# Autodesk Inventor assembly: FinalGantry
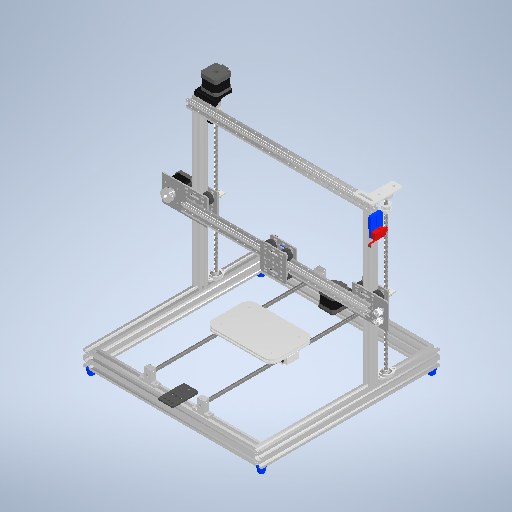
[picture p0: Inventor's stored thumbnail of the model, 512x512]
Saved by Autodesk Inventor 2025.2 (Build 292293000, 293)
## iProperties
Created: 2025-07-17
Part Number: FinalGantry
Document SubType Name: Assembly
Designer: Simon
Author: Simon
## Documents named in this file (34)
- C:\Users\Simon\Projects\Hydrogel-3D-Printer\Hardware\Bioprinter Machine Design\Final System\Final Gantry\FinalGantry.iam
- C:\Users\Simon\Projects\Hydrogel-3D-Printer\Hardware\Bioprinter Machine Design\Final System\Final Gantry\2040_AluminimProfile_410.ipt
- C:\Users\Simon\Projects\Hydrogel-3D-Printer\Hardware\Bioprinter Machine Design\Final System\Final Gantry\2040_AluminimProfile_450.ipt
- C:\Users\Simon\Projects\Hydrogel-3D-Printer\Hardware\Bioprinter Machine Design\Final System\Final Gantry\2020_AluminiumProfile_380.ipt
- C:\Users\Simon\Projects\Hydrogel-3D-Printer\Hardware\Bioprinter Machine Design\Final System\Final Gantry\2020_AluminiumProfile_465.ipt
- C:\Users\Simon\Projects\Hydrogel-3D-Printer\Hardware\Bioprinter Machine Design\PartsFolder\bracket nema 17.ipt
- C:\Users\Simon\Projects\Hydrogel-3D-Printer\Hardware\Bioprinter Machine Design\PartsFolder\Pillow Block Bearing 1\Zinc Alloy Pillow Block Flange Bearing KFL08 ID-8mm.iam
- C:\Users\Simon\Projects\Hydrogel-3D-Printer\Hardware\Bioprinter Machine Design\PartsFolder\Stepper_17HS4401.ipt
- C:\Users\Simon\Projects\Hydrogel-3D-Printer\Hardware\Bioprinter Machine Design\PartsFolder\Flexible Coupling 5,8.ipt
- C:\Users\Simon\Projects\Hydrogel-3D-Printer\Hardware\Bioprinter Machine Design\Final System\Final Gantry\TR8x8-4_LeadScrew_385.ipt
- C:\Users\Simon\Projects\Hydrogel-3D-Printer\Hardware\Bioprinter Machine Design\PartsFolder\TR8x8-4_Nut.ipt
- C:\Users\Simon\Projects\Hydrogel-3D-Printer\Hardware\Bioprinter Machine Design\PartsFolder\Nema 17 Flat Mount.ipt
- C:\Users\Simon\Projects\Hydrogel-3D-Printer\Hardware\Bioprinter Machine Design\PartsFolder\GT2_20T_5.ipt
- C:\Users\Simon\Projects\Hydrogel-3D-Printer\Hardware\Bioprinter Machine Design\PartsFolder\SK8_LinearShaftSupport.ipt
- C:\Users\Simon\Projects\Hydrogel-3D-Printer\Hardware\Bioprinter Machine Design\Final System\Final Gantry\SteelShaft_444mm.ipt
- C:\Users\Simon\Projects\Hydrogel-3D-Printer\Hardware\Bioprinter Machine Design\PartsFolder\SC8UU\SC8UU.iam
- C:\Users\Simon\Projects\Hydrogel-3D-Printer\Hardware\Bioprinter Machine Design\PartsFolder\POM Wheel v2.ipt
- C:\Users\Simon\Projects\Hydrogel-3D-Printer\Hardware\Bioprinter Machine Design\PartsFolder\Carriage Plate v1.ipt
- C:\Users\Simon\Projects\Hydrogel-3D-Printer\Hardware\Bioprinter Machine Design\PartsFolder\Spacer v2.ipt
- C:\Users\Simon\Projects\Hydrogel-3D-Printer\Hardware\Bioprinter Machine Design\Final System\Final Gantry\2020_AluminiumProfile_460.ipt
- C:\Users\Simon\Projects\Hydrogel-3D-Printer\Hardware\Bioprinter Machine Design\Final System\Final Gantry\LeadCarriageConnector.ipt
- C:\Users\Simon\Projects\Hydrogel-3D-Printer\Hardware\Bioprinter Machine Design\Final System\Final Gantry\CarriagePlate_Motor.ipt
- C:\Users\Simon\Projects\Hydrogel-3D-Printer\Hardware\Bioprinter Machine Design\Final System\Final Gantry\CarriagePlate_Idler.ipt
- C:\Users\Simon\Projects\Hydrogel-3D-Printer\Hardware\Bioprinter Machine Design\PartsFolder\GT2_20T_Toothed_Idler_5.ipt
- C:\Users\Simon\Projects\Hydrogel-3D-Printer\Hardware\Bioprinter Machine Design\PartsFolder\Idler Pulley Plate.ipt
- C:\Users\Simon\Projects\Hydrogel-3D-Printer\Hardware\Bioprinter Machine Design\Final System\Final Gantry\BedHeatSink.ipt
- C:\Users\Simon\Projects\Hydrogel-3D-Printer\Hardware\Bioprinter Machine Design\PartsFolder\PeltierTEC1_12706.ipt
- C:\Users\Simon\Projects\Hydrogel-3D-Printer\Hardware\Bioprinter Machine Design\Final System\Final Gantry\ColdPlate.ipt
- C:\Users\Simon\Projects\Hydrogel-3D-Printer\Hardware\Bioprinter Machine Design\Final System\Final Gantry\LeadScrewEndMount.ipt
- C:\Users\Simon\Projects\Hydrogel-3D-Printer\Hardware\Bioprinter Machine Design\PartsFolder\GT2_36T_5.ipt
- C:\Users\Simon\Projects\Hydrogel-3D-Printer\Hardware\Bioprinter Machine Design\PartsFolder\GT2_30T_8.ipt
- C:\Users\Simon\Projects\Hydrogel-3D-Printer\Hardware\Bioprinter Machine Design\Gantry Concept 3\LimitSwitch.ipt
- C:\Users\Simon\Projects\Hydrogel-3D-Printer\Hardware\Bioprinter Machine Design\PartsFolder\Limit Switch\LimitSwitchPart.iam
- C:\Users\Simon\Projects\Hydrogel-3D-Printer\Hardware\Bioprinter Machine Design\Final System\Final Gantry\PrinterFeet.ipt
## Components (96 placed, 33 different names)
1. 2040_AluminimProfile_410:1 — Mate:6, Mate:7, Flush:1, Mate:10, Mate:38, Mate:39, Flush:16, Flush:17, Flush:56, Mate:146, Flush:61, Mate:150, Mate:179, Mate:185
2. 2040_AluminimProfile_450:1 — Mate:1, Mate:2, Mate:4, Mate:7, Flush:1, Mate:9, Flush:2, Mate:11, Flush:3, Mate:14, Mate:16, Angle:2, Mate:183, Mate:186
3. 2040_AluminimProfile_410:2 — Mate:8, Mate:9, Flush:2, Mate:31, Mate:32, Mate:36, Mate:37, Flush:14, Flush:15, Mate:182, Mate:184
4. 2040_AluminimProfile_450:2 — Mate:3, Mate:5, Mate:10, Mate:12, Flush:4, Mate:15, Mate:17, Angle:3, Flush:51, Flush:57, Mate:180, Mate:181, Mate:187
5. 2020_AluminiumProfile_380:1 — Mate:11, Flush:3, Flush:7, Mate:82, Flush:41
6. 2020_AluminiumProfile_380:2 — Mate:12, Flush:4, Mate:13, Flush:5, Flush:6, Mate:83, Mate:98, Flush:56, Mate:171, Flush:68
7. 2020_AluminiumProfile_465:1 — Mate:13, Flush:5, Flush:6, Flush:7, Mate:18, Flush:9, Flush:59, Mate:160, Flush:64, Flush:65
8. bracket nema 17:1 — Mate:18, Mate:19, Flush:9, Mate:20, Mate:21, Angle:1
9. Zinc Alloy Pillow Block Flange Bearing KFL08 ID-8mm:1 [sub-assembly] — Mate:14, Mate:16, Flush:8, Mate:19, Mate:23
10. Zinc Alloy Pillow Block Flange Bearing KFL08 ID-8mm:2 [sub-assembly] — Mate:15, Mate:17, Flush:8, Mate:24, Mate:145
11. Stepper_17HS4401:1 — Mate:20, Mate:21, Angle:1, Mate:22, Flush:10, Mate:25
12. Flexible Coupling 5,8:1 — Mate:22, Flush:10, Mate:170
13. TR8x8-4_LeadScrew_385:1 — Mate:23, Flush:11, Mate:25, Mate:26, Mate:169
14. TR8x8-4_LeadScrew_385:2 — Mate:24, Flush:11, Mate:27, Mate:144, Mate:168
15. TR8x8-4_Nut:1 — Mate:26, Flush:12, Angle:5, Mate:90
16. TR8x8-4_Nut:2 — Mate:27, Flush:12, Angle:4
17. Nema 17 Flat Mount:1 — Mate:31, Mate:32, Mate:33, Mate:34, Flush:60, Angle:11
18. Stepper_17HS4401:2 — Mate:33, Mate:34, Mate:35, Angle:11
19. GT2_20T_5:1 — Mate:35, Flush:62
20. SK8_LinearShaftSupport:1 — Mate:36, Flush:14, Mate:40
21. SK8_LinearShaftSupport:2 — Mate:37, Flush:15, Mate:41
22. SK8_LinearShaftSupport:3 — Mate:38, Flush:17, Mate:40, Mate:42, Flush:18
23. SK8_LinearShaftSupport:4 — Mate:39, Flush:16, Mate:41, Mate:43, Flush:19
24. SteelShaft_444mm:1 — Mate:42, Flush:18, Mate:44
25. SteelShaft_444mm:2 — Mate:43, Flush:19, Mate:45
26. SC8UU:1 [sub-assembly] — Mate:44, Angle:2, Flush:20, Flush:58, Mate:147
27. SC8UU:2 [sub-assembly] — Mate:45, Angle:3, Flush:20, Mate:143, Mate:148, Mate:149
28. POM Wheel v2:1 — Mate:54, Flush:27, Mate:62, Mate:99
29. POM Wheel v2:2 — Flush:27, Flush:28, Mate:61, Mate:82, Mate:105
30. POM Wheel v2:3 — Flush:28, Flush:29, Mate:104
31. POM Wheel v2:4 — Flush:29, Mate:103
32. Carriage Plate v1:2 — Mate:54, Mate:56, Mate:57, Mate:58, Mate:59, Mate:60, Mate:85, Mate:87, Mate:89, Flush:40, Flush:41
33. Spacer v2:1 — Flush:24, Mate:62, Mate:99
34. Spacer v2:2 — Flush:24, Flush:25, Mate:100, Mate:105, Mate:130
35. Spacer v2:3 — Flush:25, Flush:26, Mate:102
36. Spacer v2:4 — Flush:26, Mate:101, Mate:129, Mate:131
37. Spacer v2:5 — Mate:56, Flush:21
38. Spacer v2:6 — Mate:57, Flush:21, Flush:22, Mate:60, Mate:61, Mate:100
39. Spacer v2:7 — Mate:58, Flush:22, Flush:23, Mate:102, Mate:104
40. Spacer v2:8 — Mate:59, Flush:23, Mate:101, Mate:103
41. POM Wheel v2:5 — Mate:91
42. POM Wheel v2:6 — Mate:83, Mate:97
43. POM Wheel v2:7 — Mate:95
44. POM Wheel v2:8 — Mate:96
45. Carriage Plate v1:4 — Mate:84, Mate:86, Mate:88, Mate:98, Flush:40
46. Spacer v2:9 — Mate:91, Mate:137
47. Spacer v2:10 — Mate:93, Mate:138
48. Spacer v2:11 — Mate:94, Mate:95, Mate:136
49. Spacer v2:12 — Mate:92
50. Spacer v2:13
51. Spacer v2:14 — Mate:93, Mate:97
52. Spacer v2:15 — Mate:94
53. Spacer v2:16 — Mate:92, Mate:96
54. 2020_AluminiumProfile_460:1 — Flush:51, Flush:52, Flush:53, Mate:132, Flush:54
55. LeadCarriageConnector:1 — Mate:84, Mate:86, Mate:88, Angle:4
56. LeadCarriageConnector:2 — Mate:85, Mate:87, Mate:89, Angle:5, Mate:90
57. POM Wheel v2:9 — Flush:52
58. POM Wheel v2:10
59. POM Wheel v2:11
60. POM Wheel v2:12
61. Carriage Plate v1:5 — Flush:53, Mate:172, Angle:8, Mate:173
62. Spacer v2:17 — Mate:127
63. Spacer v2:18 — Mate:128
64. Spacer v2:19 — Mate:126
65. Spacer v2:20
66. Spacer v2:21
67. Spacer v2:22
68. Spacer v2:23
69. Spacer v2:24
70. Carriage Plate v1:6 — Mate:126, Mate:127, Mate:128
71. Stepper_17HS4401:3 — Mate:133, Mate:134, Angle:6, Mate:167
72. CarriagePlate_Motor:1 — Mate:129, Mate:130, Mate:131, Mate:132, Flush:54, Mate:133, Mate:134, Angle:6
73. CarriagePlate_Idler:1 — Mate:136, Mate:137, Mate:138, Mate:141, Mate:161, Mate:165, Mate:166
74. GT2_20T_Toothed_Idler_5:1 — Mate:142, Mate:162, Flush:66
75. Spacer v2:25 — Mate:141, Mate:142, Mate:161, Mate:162
76. Zinc Alloy Pillow Block Flange Bearing KFL08 ID-8mm:3 [sub-assembly] — Mate:144, Flush:59, Mate:145
77. Idler Pulley Plate:1 — Mate:146, Flush:60, Flush:61, Mate:150, Mate:151, Mate:157, Mate:158
78. BedHeatSink:1 — Mate:147, Mate:148, Mate:149, Mate:152, Angle:7, Mate:153, Flush:63, Mate:154, Mate:155
79. GT2_20T_Toothed_Idler_5:2 — Mate:151, Flush:62, Mate:159
80. PeltierTEC1_12706:1 — Mate:152, Angle:7, Mate:153, Flush:63, Mate:156
81. ColdPlate:1 — Mate:154, Mate:155, Mate:156
82. Spacer v2:26 — Mate:157, Mate:158, Mate:159
83. LeadScrewEndMount:1 — Mate:160, Flush:64, Flush:65, Mate:176
84. GT2_20T_Toothed_Idler_5:3 — Mate:166
85. Spacer v2:27 — Mate:165
86. GT2_36T_5:1 — Mate:167, Flush:66
87. GT2_30T_8:1 — Mate:169, Flush:67, Mate:170
88. GT2_30T_8:2 — Mate:168, Flush:67
89. LimitSwitch:1 — Mate:171, Flush:68, Mate:176, Mate:177, Angle:10, Mate:178
90. LimitSwitch:2 — Mate:172, Angle:8, Mate:173, Mate:174, Angle:9, Mate:175
91. LimitSwitchPart:1 [sub-assembly] — Mate:177, Angle:10, Mate:178
92. LimitSwitchPart:2 [sub-assembly] — Mate:174, Angle:9, Mate:175
93. PrinterFeet:1 — Flush:70, Mate:183, Mate:184
94. PrinterFeet:2 — Flush:69, Flush:70, Mate:185, Mate:186
95. PrinterFeet:3 — Flush:69, Flush:71, Mate:181, Mate:182
96. PrinterFeet:4 — Flush:71, Mate:179, Mate:180, Mate:187
## Relationships (235: Mate 156, Flush 68, Angle 11)
- Mate:1: 2040_AluminimProfile_450:1
- Mate:2: 2040_AluminimProfile_450:1
- Mate:3: 2040_AluminimProfile_450:2
- Mate:4: 2040_AluminimProfile_450:1
- Mate:5: 2040_AluminimProfile_450:2
- Mate:6: 2040_AluminimProfile_410:1
- Mate:7: 2040_AluminimProfile_410:1 ↔ 2040_AluminimProfile_450:1
- Flush:1: 2040_AluminimProfile_410:1 ↔ 2040_AluminimProfile_450:1
- Mate:8: 2040_AluminimProfile_410:2
- Mate:9: 2040_AluminimProfile_450:1 ↔ 2040_AluminimProfile_410:2
- Flush:2: 2040_AluminimProfile_450:1 ↔ 2040_AluminimProfile_410:2
- Mate:10: 2040_AluminimProfile_410:1 ↔ 2040_AluminimProfile_450:2
- Mate:11: 2040_AluminimProfile_450:1 ↔ 2020_AluminiumProfile_380:1
- Mate:12: 2040_AluminimProfile_450:2 ↔ 2020_AluminiumProfile_380:2
- Flush:3: 2040_AluminimProfile_450:1 ↔ 2020_AluminiumProfile_380:1
- Flush:4: 2040_AluminimProfile_450:2 ↔ 2020_AluminiumProfile_380:2
- Mate:13: 2020_AluminiumProfile_380:2 ↔ 2020_AluminiumProfile_465:1
- Flush:5: 2020_AluminiumProfile_380:2 ↔ 2020_AluminiumProfile_465:1
- Flush:6: 2020_AluminiumProfile_380:2 ↔ 2020_AluminiumProfile_465:1
- Flush:7: 2020_AluminiumProfile_380:1 ↔ 2020_AluminiumProfile_465:1
- Mate:14: 2040_AluminimProfile_450:1 ↔ Zinc Alloy Pillow Block Flange Bearing KFL08 ID-8mm:1
- Mate:15: 2040_AluminimProfile_450:2 ↔ Zinc Alloy Pillow Block Flange Bearing KFL08 ID-8mm:2
- Mate:16: 2040_AluminimProfile_450:1 ↔ Zinc Alloy Pillow Block Flange Bearing KFL08 ID-8mm:1
- Mate:17: 2040_AluminimProfile_450:2 ↔ Zinc Alloy Pillow Block Flange Bearing KFL08 ID-8mm:2
- Flush:8: Zinc Alloy Pillow Block Flange Bearing KFL08 ID-8mm:1 ↔ Zinc Alloy Pillow Block Flange Bearing KFL08 ID-8mm:2
- Mate:18: 2020_AluminiumProfile_465:1 ↔ bracket nema 17:1
- Mate:19: bracket nema 17:1 ↔ Zinc Alloy Pillow Block Flange Bearing KFL08 ID-8mm:1
- Flush:9 (-10 mm): 2020_AluminiumProfile_465:1 ↔ bracket nema 17:1
- Mate:20: bracket nema 17:1 ↔ Stepper_17HS4401:1
- Mate:21: bracket nema 17:1 ↔ Stepper_17HS4401:1
- Angle:1 (0 deg): bracket nema 17:1 ↔ Stepper_17HS4401:1
- Mate:22: Stepper_17HS4401:1 ↔ Flexible Coupling 5,8:1
- Flush:10 (5 mm): Stepper_17HS4401:1 ↔ Flexible Coupling 5,8:1
- Mate:23: Zinc Alloy Pillow Block Flange Bearing KFL08 ID-8mm:1 ↔ TR8x8-4_LeadScrew_385:1
- Mate:24: Zinc Alloy Pillow Block Flange Bearing KFL08 ID-8mm:2 ↔ TR8x8-4_LeadScrew_385:2
- Flush:11: TR8x8-4_LeadScrew_385:1 ↔ TR8x8-4_LeadScrew_385:2
- Mate:25: Stepper_17HS4401:1 ↔ TR8x8-4_LeadScrew_385:1
- Mate:26: TR8x8-4_LeadScrew_385:1 ↔ TR8x8-4_Nut:1
- Mate:27: TR8x8-4_LeadScrew_385:2 ↔ TR8x8-4_Nut:2
- Flush:12: TR8x8-4_Nut:1 ↔ TR8x8-4_Nut:2
- Mate:31: 2040_AluminimProfile_410:2 ↔ Nema 17 Flat Mount:1
- Mate:32: 2040_AluminimProfile_410:2 ↔ Nema 17 Flat Mount:1
- Mate:33: Nema 17 Flat Mount:1 ↔ Stepper_17HS4401:2
- Mate:34: Nema 17 Flat Mount:1 ↔ Stepper_17HS4401:2
- Mate:35: Stepper_17HS4401:2 ↔ GT2_20T_5:1
- Mate:36: 2040_AluminimProfile_410:2 ↔ SK8_LinearShaftSupport:1
- Mate:37: 2040_AluminimProfile_410:2 ↔ SK8_LinearShaftSupport:2
- Mate:38: 2040_AluminimProfile_410:1 ↔ SK8_LinearShaftSupport:3
- Mate:39: 2040_AluminimProfile_410:1 ↔ SK8_LinearShaftSupport:4
- Flush:14: 2040_AluminimProfile_410:2 ↔ SK8_LinearShaftSupport:1
- Flush:15: 2040_AluminimProfile_410:2 ↔ SK8_LinearShaftSupport:2
- Flush:16: 2040_AluminimProfile_410:1 ↔ SK8_LinearShaftSupport:4
- Flush:17: 2040_AluminimProfile_410:1 ↔ SK8_LinearShaftSupport:3
- Mate:40: SK8_LinearShaftSupport:1 ↔ SK8_LinearShaftSupport:3
- Mate:41: SK8_LinearShaftSupport:2 ↔ SK8_LinearShaftSupport:4
- Mate:42: SK8_LinearShaftSupport:3 ↔ SteelShaft_444mm:1
- Mate:43: SK8_LinearShaftSupport:4 ↔ SteelShaft_444mm:2
- Flush:18: SK8_LinearShaftSupport:3 ↔ SteelShaft_444mm:1
- Flush:19: SK8_LinearShaftSupport:4 ↔ SteelShaft_444mm:2
- Mate:44: SteelShaft_444mm:1 ↔ SC8UU:1
- Mate:45: SteelShaft_444mm:2 ↔ SC8UU:2
- Angle:2 (0 deg): 2040_AluminimProfile_450:1 ↔ SC8UU:1
- Angle:3 (0 deg): 2040_AluminimProfile_450:2 ↔ SC8UU:2
- Flush:20: SC8UU:1 ↔ SC8UU:2
- Mate:54: POM Wheel v2:1 ↔ Carriage Plate v1:2
- Mate:56: Carriage Plate v1:2 ↔ Spacer v2:5
- Mate:57: Carriage Plate v1:2 ↔ Spacer v2:6
- Mate:58: Carriage Plate v1:2 ↔ Spacer v2:7
- Mate:59: Carriage Plate v1:2 ↔ Spacer v2:8
- Flush:21: Spacer v2:5 ↔ Spacer v2:6
- Flush:22: Spacer v2:6 ↔ Spacer v2:7
- Flush:23: Spacer v2:7 ↔ Spacer v2:8
- Mate:60: Carriage Plate v1:2 ↔ Spacer v2:6
- Flush:24: Spacer v2:1 ↔ Spacer v2:2
- Flush:25: Spacer v2:2 ↔ Spacer v2:3
- Flush:26: Spacer v2:3 ↔ Spacer v2:4
- Flush:27: POM Wheel v2:1 ↔ POM Wheel v2:2
- Flush:28: POM Wheel v2:2 ↔ POM Wheel v2:3
- Flush:29: POM Wheel v2:3 ↔ POM Wheel v2:4
- Mate:61: POM Wheel v2:2 ↔ Spacer v2:6
- Mate:62: POM Wheel v2:1 ↔ Spacer v2:1
- [Mate]: POM Wheel v2:5 ↔ Carriage Plate v1:4
- [Mate]: Carriage Plate v1:4 ↔ Spacer v2:13
- [Mate]: Carriage Plate v1:4 ↔ Spacer v2:14
- [Mate]: Carriage Plate v1:4 ↔ Spacer v2:15
- [Mate]: Carriage Plate v1:4 ↔ Spacer v2:16
- [Flush]: Spacer v2:13 ↔ Spacer v2:14
- [Flush]: Spacer v2:14 ↔ Spacer v2:15
- [Flush]: Spacer v2:15 ↔ Spacer v2:16
- [Mate]: Carriage Plate v1:4 ↔ Spacer v2:14
- [Flush]: Spacer v2:9 ↔ Spacer v2:10
- [Flush]: Spacer v2:10 ↔ Spacer v2:11
- [Flush]: Spacer v2:11 ↔ Spacer v2:12
- [Flush]: POM Wheel v2:5 ↔ POM Wheel v2:6
- [Flush]: POM Wheel v2:6 ↔ POM Wheel v2:7
- [Flush]: POM Wheel v2:7 ↔ POM Wheel v2:8
- [Mate]: POM Wheel v2:6 ↔ Spacer v2:14
- [Mate]: POM Wheel v2:5 ↔ Spacer v2:9
- Mate:82: 2020_AluminiumProfile_380:1 ↔ POM Wheel v2:2
- Mate:83: 2020_AluminiumProfile_380:2 ↔ POM Wheel v2:6
- Mate:84: Carriage Plate v1:4 ↔ LeadCarriageConnector:1
- Mate:85: Carriage Plate v1:2 ↔ LeadCarriageConnector:2
- Mate:86: Carriage Plate v1:4 ↔ LeadCarriageConnector:1
- Mate:87: Carriage Plate v1:2 ↔ LeadCarriageConnector:2
- Mate:88: Carriage Plate v1:4 ↔ LeadCarriageConnector:1
- Mate:89: Carriage Plate v1:2 ↔ LeadCarriageConnector:2
- Angle:4 (0 deg): TR8x8-4_Nut:2 ↔ LeadCarriageConnector:1
- Angle:5 (0 deg): TR8x8-4_Nut:1 ↔ LeadCarriageConnector:2
- Mate:90: TR8x8-4_Nut:1 ↔ LeadCarriageConnector:2
- Mate:91: POM Wheel v2:5 ↔ Spacer v2:9
- Mate:92: Spacer v2:12 ↔ Spacer v2:16
- Mate:93: Spacer v2:10 ↔ Spacer v2:14
- Mate:94: Spacer v2:11 ↔ Spacer v2:15
- Mate:95: POM Wheel v2:7 ↔ Spacer v2:11
- Mate:96: POM Wheel v2:8 ↔ Spacer v2:16
- Mate:97: POM Wheel v2:6 ↔ Spacer v2:14
- Mate:98: 2020_AluminiumProfile_380:2 ↔ Carriage Plate v1:4
- Flush:40: Carriage Plate v1:2 ↔ Carriage Plate v1:4
- Mate:99: POM Wheel v2:1 ↔ Spacer v2:1
- Mate:100: Spacer v2:2 ↔ Spacer v2:6
- Mate:101: Spacer v2:4 ↔ Spacer v2:8
- Mate:102: Spacer v2:3 ↔ Spacer v2:7
- Mate:103: POM Wheel v2:4 ↔ Spacer v2:8
- Mate:104: POM Wheel v2:3 ↔ Spacer v2:7
- Mate:105: POM Wheel v2:2 ↔ Spacer v2:2
- Flush:41: 2020_AluminiumProfile_380:1 ↔ Carriage Plate v1:2
- [Mate]: POM Wheel v2:9 ↔ Carriage Plate v1:5
- [Mate]: Carriage Plate v1:5 ↔ Spacer v2:21
- [Mate]: Carriage Plate v1:5 ↔ Spacer v2:22
- [Mate]: Carriage Plate v1:5 ↔ Spacer v2:23
- [Mate]: Carriage Plate v1:5 ↔ Spacer v2:24
- [Flush]: Spacer v2:21 ↔ Spacer v2:22
- [Flush]: Spacer v2:22 ↔ Spacer v2:23
- [Flush]: Spacer v2:23 ↔ Spacer v2:24
- [Mate]: Carriage Plate v1:5 ↔ Spacer v2:22
- [Flush]: Spacer v2:17 ↔ Spacer v2:18
- [Flush]: Spacer v2:18 ↔ Spacer v2:19
- [Flush]: Spacer v2:19 ↔ Spacer v2:20
- [Flush]: POM Wheel v2:9 ↔ POM Wheel v2:10
- [Flush]: POM Wheel v2:10 ↔ POM Wheel v2:11
- [Flush]: POM Wheel v2:11 ↔ POM Wheel v2:12
- [Mate]: POM Wheel v2:10 ↔ Spacer v2:22
- [Mate]: POM Wheel v2:9 ↔ Spacer v2:17
- [Mate]: POM Wheel v2:9 ↔ Spacer v2:17
- [Mate]: Spacer v2:18 ↔ Spacer v2:22
- [Mate]: Spacer v2:20 ↔ Spacer v2:24
- [Mate]: Spacer v2:19 ↔ Spacer v2:23
- [Mate]: POM Wheel v2:12 ↔ Spacer v2:24
- [Mate]: POM Wheel v2:11 ↔ Spacer v2:23
- [Mate]: POM Wheel v2:10 ↔ Spacer v2:18
- Flush:51 (225 mm): 2040_AluminimProfile_450:2 ↔ 2020_AluminiumProfile_460:1
- Flush:52: 2020_AluminiumProfile_460:1 ↔ POM Wheel v2:9
- Flush:53: 2020_AluminiumProfile_460:1 ↔ Carriage Plate v1:5
- Mate:126: Spacer v2:19 ↔ Carriage Plate v1:6
- Mate:127: Spacer v2:17 ↔ Carriage Plate v1:6
- Mate:128: Spacer v2:18 ↔ Carriage Plate v1:6
- Mate:129: Spacer v2:4 ↔ CarriagePlate_Motor:1
- Mate:130: Spacer v2:2 ↔ CarriagePlate_Motor:1
- Mate:131: Spacer v2:4 ↔ CarriagePlate_Motor:1
- Mate:132: 2020_AluminiumProfile_460:1 ↔ CarriagePlate_Motor:1
- Flush:54: 2020_AluminiumProfile_460:1 ↔ CarriagePlate_Motor:1
- Mate:133: Stepper_17HS4401:3 ↔ CarriagePlate_Motor:1
- Mate:134: Stepper_17HS4401:3 ↔ CarriagePlate_Motor:1
- Angle:6 (0 deg): Stepper_17HS4401:3 ↔ CarriagePlate_Motor:1
- Mate:136: Spacer v2:11 ↔ CarriagePlate_Idler:1
- Mate:137: Spacer v2:9 ↔ CarriagePlate_Idler:1
- Mate:138: Spacer v2:10 ↔ CarriagePlate_Idler:1
- Mate:141: CarriagePlate_Idler:1 ↔ Spacer v2:25
- Mate:142: GT2_20T_Toothed_Idler_5:1 ↔ Spacer v2:25
- Flush:56 (275 mm): 2040_AluminimProfile_410:1 ↔ 2020_AluminiumProfile_380:2
- Flush:57 (-225 mm): 2040_AluminimProfile_450:2
- Mate:143 (50 mm): SC8UU:2
- Flush:58 (50 mm): SC8UU:1
- Mate:144: TR8x8-4_LeadScrew_385:2 ↔ Zinc Alloy Pillow Block Flange Bearing KFL08 ID-8mm:3
- Flush:59: 2020_AluminiumProfile_465:1 ↔ Zinc Alloy Pillow Block Flange Bearing KFL08 ID-8mm:3
- Mate:145: Zinc Alloy Pillow Block Flange Bearing KFL08 ID-8mm:2 ↔ Zinc Alloy Pillow Block Flange Bearing KFL08 ID-8mm:3
- Mate:146: 2040_AluminimProfile_410:1 ↔ Idler Pulley Plate:1
- Flush:60: Nema 17 Flat Mount:1 ↔ Idler Pulley Plate:1
- Mate:147: SC8UU:1 ↔ BedHeatSink:1
- Mate:148: SC8UU:2 ↔ BedHeatSink:1
- Mate:149: SC8UU:2 ↔ BedHeatSink:1
- Flush:61: 2040_AluminimProfile_410:1 ↔ Idler Pulley Plate:1
- Mate:150: 2040_AluminimProfile_410:1 ↔ Idler Pulley Plate:1
- Mate:151: Idler Pulley Plate:1 ↔ GT2_20T_Toothed_Idler_5:2
- Flush:62: GT2_20T_5:1 ↔ GT2_20T_Toothed_Idler_5:2
- Mate:152: BedHeatSink:1 ↔ PeltierTEC1_12706:1
- Angle:7 (0 deg): BedHeatSink:1 ↔ PeltierTEC1_12706:1
- Mate:153: BedHeatSink:1 ↔ PeltierTEC1_12706:1
- Flush:63: BedHeatSink:1 ↔ PeltierTEC1_12706:1
- Mate:154: BedHeatSink:1 ↔ ColdPlate:1
- Mate:155: BedHeatSink:1 ↔ ColdPlate:1
- Mate:156: PeltierTEC1_12706:1 ↔ ColdPlate:1
- Mate:157: Idler Pulley Plate:1 ↔ Spacer v2:26
- Mate:158: Idler Pulley Plate:1 ↔ Spacer v2:26
- Mate:159: GT2_20T_Toothed_Idler_5:2 ↔ Spacer v2:26
- Mate:160: 2020_AluminiumProfile_465:1 ↔ LeadScrewEndMount:1
- Flush:64: 2020_AluminiumProfile_465:1 ↔ LeadScrewEndMount:1
- Flush:65 (-4 mm): 2020_AluminiumProfile_465:1 ↔ LeadScrewEndMount:1
- Mate:161: CarriagePlate_Idler:1 ↔ Spacer v2:25
- Mate:162: GT2_20T_Toothed_Idler_5:1 ↔ Spacer v2:25
- [Mate]: GT2_20T_Toothed_Idler_5:3 ↔ Spacer v2:27
- [Mate]: GT2_20T_Toothed_Idler_5:3 ↔ Spacer v2:27
- Mate:165: CarriagePlate_Idler:1 ↔ Spacer v2:27
- Mate:166: CarriagePlate_Idler:1 ↔ GT2_20T_Toothed_Idler_5:3
- Mate:167: Stepper_17HS4401:3 ↔ GT2_36T_5:1
- Flush:66: GT2_20T_Toothed_Idler_5:1 ↔ GT2_36T_5:1
- Mate:168: TR8x8-4_LeadScrew_385:2 ↔ GT2_30T_8:2
- Mate:169: TR8x8-4_LeadScrew_385:1 ↔ GT2_30T_8:1
- Flush:67: GT2_30T_8:1 ↔ GT2_30T_8:2
- Mate:170: Flexible Coupling 5,8:1 ↔ GT2_30T_8:1
- Mate:171: 2020_AluminiumProfile_380:2 ↔ LimitSwitch:1
- Mate:172: Carriage Plate v1:5 ↔ LimitSwitch:2
- Angle:8 (0 deg): Carriage Plate v1:5 ↔ LimitSwitch:2
- Mate:173: Carriage Plate v1:5 ↔ LimitSwitch:2
- Mate:174: LimitSwitch:2 ↔ LimitSwitchPart:2
- Angle:9 (0 deg): LimitSwitch:2 ↔ LimitSwitchPart:2
- Mate:175: LimitSwitch:2 ↔ LimitSwitchPart:2
- Flush:68: 2020_AluminiumProfile_380:2 ↔ LimitSwitch:1
- Mate:176 (20 mm): LeadScrewEndMount:1 ↔ LimitSwitch:1
- Mate:177: LimitSwitch:1 ↔ LimitSwitchPart:1
- Angle:10 (0 deg): LimitSwitch:1 ↔ LimitSwitchPart:1
- Mate:178: LimitSwitch:1 ↔ LimitSwitchPart:1
- Flush:69: PrinterFeet:2 ↔ PrinterFeet:3
- Flush:70: PrinterFeet:1 ↔ PrinterFeet:2
- Flush:71: PrinterFeet:3 ↔ PrinterFeet:4
- Mate:179: 2040_AluminimProfile_410:1 ↔ PrinterFeet:4
- Mate:180: 2040_AluminimProfile_450:2 ↔ PrinterFeet:4
- Mate:181: 2040_AluminimProfile_450:2 ↔ PrinterFeet:3
- Mate:182: 2040_AluminimProfile_410:2 ↔ PrinterFeet:3
- Mate:183: 2040_AluminimProfile_450:1 ↔ PrinterFeet:1
- Mate:184: 2040_AluminimProfile_410:2 ↔ PrinterFeet:1
- Mate:185: 2040_AluminimProfile_410:1 ↔ PrinterFeet:2
- Mate:186: 2040_AluminimProfile_450:1 ↔ PrinterFeet:2
- Mate:187: 2040_AluminimProfile_450:2 ↔ PrinterFeet:4
- Angle:11 (0 deg): Nema 17 Flat Mount:1 ↔ Stepper_17HS4401:2
## Named parameters: d95_d80 = 0 mm, d96_d81 = 0 mm, d97_d82 = 0 mm, d98_d83 = 0 mm, d99_d84 = 0 mm, d100_d85 = 0 mm, d101_d86 = 0 mm, d102_d87 = 0 mm, d103_d88 = 0 mm, d104_d89 = 0 mm, d105_d90 = 0 mm, d106_d91 = 0 mm, d107_d92 = 0 mm, d108_d93 = 0 mm, d118_d76 = 0 mm, d120_d78 = 0 mm, d121_d79 = 0 mm, d157_d76 = 0 mm, d158_d78 = 0 mm, d159_d79 = 0 mm, d160_d80 = 0 mm, d161_d81 = 0 mm, d162_d82 = 0 mm, d163_d83 = 0 mm, d164_d84 = 0 mm, d165_d85 = 0 mm, d166_d86 = 0 mm, d167_d87 = 0 mm, d168_d88 = 0 mm, d169_d89 = 0 mm, d170_d90 = 0 mm, d171_d91 = 0 mm, d172_d92 = 0 mm, d173_d93 = 0 mm, d174_d145 = 0 mm, d175_d146 = 0 mm, d176_d147 = 0 mm, d177_d148 = 0 mm, d178_d149 = 0 mm, d179_d150 = 0 mm, d180_d151 = 0 mm, d238_d206 = 0 mm, d239_d237 = 0 mm
